# Autodesk Inventor assembly: coil_driver
(part 2 of 3)
- C:\Users\nfitch\Desktop\repos\Imperial\CCMCircuits\CCM_0008_Coil_Driver\cad\RESC1608X446.ipt
- C:\Users\nfitch\Desktop\repos\Imperial\CCMCircuits\CCM_0008_Coil_Driver\cad\RESC1608X447.ipt
- C:\Users\nfitch\Desktop\repos\Imperial\CCMCircuits\CCM_0008_Coil_Driver\cad\RESC1608X448.ipt
- C:\Users\nfitch\Desktop\repos\Imperial\CCMCircuits\CCM_0008_Coil_Driver\cad\RESC1608X449.ipt
- C:\Users\nfitch\Desktop\repos\Imperial\CCMCircuits\CCM_0008_Coil_Driver\cad\RESC1608X450.ipt
- C:\Users\nfitch\Desktop\repos\Imperial\CCMCircuits\CCM_0008_Coil_Driver\cad\RESC1608X451.ipt
- C:\Users\nfitch\Desktop\repos\Imperial\CCMCircuits\CCM_0008_Coil_Driver\cad\RESC1608X452.ipt
- C:\Users\nfitch\Desktop\repos\Imperial\CCMCircuits\CCM_0008_Coil_Driver\cad\RESC1608X453.ipt
- C:\Users\nfitch\Desktop\repos\Imperial\CCMCircuits\CCM_0008_Coil_Driver\cad\RESC1608X454.ipt
- C:\Users\nfitch\Desktop\repos\Imperial\CCMCircuits\CCM_0008_Coil_Driver\cad\RESC1608X455.ipt
- C:\Users\nfitch\Desktop\repos\Imperial\CCMCircuits\CCM_0008_Coil_Driver\cad\RESC1608X456.ipt
- C:\Users\nfitch\Desktop\repos\Imperial\CCMCircuits\CCM_0008_Coil_Driver\cad\RESC1608X457.ipt
- C:\Users\nfitch\Desktop\repos\Imperial\CCMCircuits\CCM_0008_Coil_Driver\cad\RESC1608X458.ipt
- C:\Users\nfitch\Desktop\repos\Imperial\CCMCircuits\CCM_0008_Coil_Driver\cad\RESC1608X459.ipt
- C:\Users\nfitch\Desktop\repos\Imperial\CCMCircuits\CCM_0008_Coil_Driver\cad\RESC1608X460.ipt
- C:\Users\nfitch\Desktop\repos\Imperial\CCMCircuits\CCM_0008_Coil_Driver\cad\RESC1608X461.ipt
- C:\Users\nfitch\Desktop\repos\Imperial\CCMCircuits\CCM_0008_Coil_Driver\cad\RESC1608X462.ipt
- C:\Users\nfitch\Desktop\repos\Imperial\CCMCircuits\CCM_0008_Coil_Driver\cad\RESC1608X463.ipt
- C:\Users\nfitch\Desktop\repos\Imperial\CCMCircuits\CCM_0008_Coil_Driver\cad\RESC1608X464.ipt
- C:\Users\nfitch\Desktop\repos\Imperial\CCMCircuits\CCM_0008_Coil_Driver\cad\RESC1608X465.ipt
- C:\Users\nfitch\Desktop\repos\Imperial\CCMCircuits\CCM_0008_Coil_Driver\cad\RESC1608X466.ipt
- C:\Users\nfitch\Desktop\repos\Imperial\CCMCircuits\CCM_0008_Coil_Driver\cad\RESC1608X467.ipt
- C:\Users\nfitch\Desktop\repos\Imperial\CCMCircuits\CCM_0008_Coil_Driver\cad\RESC1608X468.ipt
- C:\Users\nfitch\Desktop\repos\Imperial\CCMCircuits\CCM_0008_Coil_Driver\cad\RESC1608X469.ipt
- C:\Users\nfitch\Desktop\repos\Imperial\CCMCircuits\CCM_0008_Coil_Driver\cad\RESC1608X470.ipt
- C:\Users\nfitch\Desktop\repos\Imperial\CCMCircuits\CCM_0008_Coil_Driver\cad\RESC1608X471.ipt
- C:\Users\nfitch\Desktop\repos\Imperial\CCMCircuits\CCM_0008_Coil_Driver\cad\RESC1608X472.ipt
- C:\Users\nfitch\Desktop\repos\Imperial\CCMCircuits\CCM_0008_Coil_Driver\cad\RESC1608X473.ipt
- C:\Users\nfitch\Desktop\repos\Imperial\CCMCircuits\CCM_0008_Coil_Driver\cad\RESC1608X474.ipt
- C:\Users\nfitch\Desktop\repos\Imperial\CCMCircuits\CCM_0008_Coil_Driver\cad\RESC1608X475.ipt
- C:\Users\nfitch\Desktop\repos\Imperial\CCMCircuits\CCM_0008_Coil_Driver\cad\RESC1608X476.ipt
- C:\Users\nfitch\Desktop\repos\Imperial\CCMCircuits\CCM_0008_Coil_Driver\cad\RESC1608X477.ipt
- C:\Users\nfitch\Desktop\repos\Imperial\CCMCircuits\CCM_0008_Coil_Driver\cad\RESC1608X478.ipt
- C:\Users\nfitch\Desktop\repos\Imperial\CCMCircuits\CCM_0008_Coil_Driver\cad\RESC1608X479.ipt
- C:\Users\nfitch\Desktop\repos\Imperial\CCMCircuits\CCM_0008_Coil_Driver\cad\RESC1608X480.ipt
- C:\Users\nfitch\Desktop\repos\Imperial\CCMCircuits\CCM_0008_Coil_Driver\cad\RESC1608X481.ipt
- C:\Users\nfitch\Desktop\repos\Imperial\CCMCircuits\CCM_0008_Coil_Driver\cad\RESC1608X482.ipt
- C:\Users\nfitch\Desktop\repos\Imperial\CCMCircuits\CCM_0008_Coil_Driver\cad\RESC1608X483.ipt
- C:\Users\nfitch\Desktop\repos\Imperial\CCMCircuits\CCM_0008_Coil_Driver\cad\RESC1608X484.ipt
- C:\Users\nfitch\Desktop\repos\Imperial\CCMCircuits\CCM_0008_Coil_Driver\cad\RESC1608X485.ipt
- C:\Users\nfitch\Desktop\repos\Imperial\CCMCircuits\CCM_0008_Coil_Driver\cad\RESC1608X486.ipt
- C:\Users\nfitch\Desktop\repos\Imperial\CCMCircuits\CCM_0008_Coil_Driver\cad\RESC1608X487.ipt
- C:\Users\nfitch\Desktop\repos\Imperial\CCMCircuits\CCM_0008_Coil_Driver\cad\RESC1608X488.ipt
- C:\Users\nfitch\Desktop\repos\Imperial\CCMCircuits\CCM_0008_Coil_Driver\cad\RESC1608X489.ipt
- C:\Users\nfitch\Desktop\repos\Imperial\CCMCircuits\CCM_0008_Coil_Driver\cad\RESC1608X490.ipt
- C:\Users\nfitch\Desktop\repos\Imperial\CCMCircuits\CCM_0008_Coil_Driver\cad\RESC1608X491.ipt
- C:\Users\nfitch\Desktop\repos\Imperial\CCMCircuits\CCM_0008_Coil_Driver\cad\RESC1608X492.ipt
- C:\Users\nfitch\Desktop\repos\Imperial\CCMCircuits\CCM_0008_Coil_Driver\cad\RESC1608X493.ipt
- C:\Users\nfitch\Desktop\repos\Imperial\CCMCircuits\CCM_0008_Coil_Driver\cad\RESC1608X494.ipt
- C:\Users\nfitch\Desktop\repos\Imperial\CCMCircuits\CCM_0008_Coil_Driver\cad\RESC1608X495.ipt
- C:\Users\nfitch\Desktop\repos\Imperial\CCMCircuits\CCM_0008_Coil_Driver\cad\RESC1608X496.ipt
- C:\Users\nfitch\Desktop\repos\Imperial\CCMCircuits\CCM_0008_Coil_Driver\cad\RESC1608X497.ipt
- C:\Users\nfitch\Desktop\repos\Imperial\CCMCircuits\CCM_0008_Coil_Driver\cad\RESC1608X498.ipt
- C:\Users\nfitch\Desktop\repos\Imperial\CCMCircuits\CCM_0008_Coil_Driver\cad\RESC1608X499.ipt
- C:\Users\nfitch\Desktop\repos\Imperial\CCMCircuits\CCM_0008_Coil_Driver\cad\RESC1608X500.ipt
- C:\Users\nfitch\Desktop\repos\Imperial\CCMCircuits\CCM_0008_Coil_Driver\cad\RESC1608X501.ipt
- C:\Users\nfitch\Desktop\repos\Imperial\CCMCircuits\CCM_0008_Coil_Driver\cad\RESC1608X502.ipt
- C:\Users\nfitch\Desktop\repos\Imperial\CCMCircuits\CCM_0008_Coil_Driver\cad\RESC1608X503.ipt
- C:\Users\nfitch\Desktop\repos\Imperial\CCMCircuits\CCM_0008_Coil_Driver\cad\RESC1608X504.ipt
- C:\Users\nfitch\Desktop\repos\Imperial\CCMCircuits\CCM_0008_Coil_Driver\cad\RESC1608X505.ipt
- C:\Users\nfitch\Desktop\repos\Imperial\CCMCircuits\CCM_0008_Coil_Driver\cad\RESC1608X506.ipt
- C:\Users\nfitch\Desktop\repos\Imperial\CCMCircuits\CCM_0008_Coil_Driver\cad\RESC1608X507.ipt
- C:\Users\nfitch\Desktop\repos\Imperial\CCMCircuits\CCM_0008_Coil_Driver\cad\RESC1608X508.ipt
- C:\Users\nfitch\Desktop\repos\Imperial\CCMCircuits\CCM_0008_Coil_Driver\cad\RESC1608X509.ipt
- C:\Users\nfitch\Desktop\repos\Imperial\CCMCircuits\CCM_0008_Coil_Driver\cad\RESC1608X510.ipt
- C:\Users\nfitch\Desktop\repos\Imperial\CCMCircuits\CCM_0008_Coil_Driver\cad\RESC1608X511.ipt
- C:\Users\nfitch\Desktop\repos\Imperial\CCMCircuits\CCM_0008_Coil_Driver\cad\RESC1608X512.ipt
- C:\Users\nfitch\Desktop\repos\Imperial\CCMCircuits\CCM_0008_Coil_Driver\cad\RESC1608X513.ipt
- C:\Users\nfitch\Desktop\repos\Imperial\CCMCircuits\CCM_0008_Coil_Driver\cad\RESC1608X514.ipt
- C:\Users\nfitch\Desktop\repos\Imperial\CCMCircuits\CCM_0008_Coil_Driver\cad\SOD3715X136.ipt
- C:\Users\nfitch\Desktop\repos\Imperial\CCMCircuits\CCM_0008_Coil_Driver\cad\SOD3715X137.ipt
- C:\Users\nfitch\Desktop\repos\Imperial\CCMCircuits\CCM_0008_Coil_Driver\cad\SOD3715X135.ipt
- C:\Users\nfitch\Desktop\repos\Imperial\CCMCircuits\CCM_0008_Coil_Driver\cad\SOT95P237X112-005.ipt
- C:\Users\nfitch\Desktop\repos\Imperial\CCMCircuits\CCM_0008_Coil_Driver\cad\SOT95P237X112-006.ipt
- C:\Users\nfitch\Desktop\repos\Imperial\CCMCircuits\CCM_0008_Coil_Driver\cad\SOT95P237X112-3.ipt
- C:\Users\nfitch\Desktop\repos\Imperial\CCMCircuits\CCM_0008_Coil_Driver\cad\SOT95P237X112-004.ipt
- C:\Users\nfitch\Desktop\repos\Imperial\CCMCircuits\CCM_0008_Coil_Driver\cad\SOD3715X138.ipt
- C:\Users\nfitch\Desktop\repos\Imperial\CCMCircuits\CCM_0008_Coil_Driver\cad\SOD3715X139.ipt
- C:\Users\nfitch\Desktop\repos\Imperial\CCMCircuits\CCM_0008_Coil_Driver\cad\SOD3715X140.ipt
- C:\Users\nfitch\Desktop\repos\Imperial\CCMCircuits\CCM_0008_Coil_Driver\cad\SOD3715X141.ipt
- C:\Users\nfitch\Desktop\repos\Imperial\CCMCircuits\CCM_0008_Coil_Driver\cad\SOD3715X142.ipt
- C:\Users\nfitch\Desktop\repos\Imperial\CCMCircuits\CCM_0008_Coil_Driver\cad\SOD3715X143.ipt
- C:\Users\nfitch\Desktop\repos\Imperial\CCMCircuits\CCM_0008_Coil_Driver\cad\SOD3715X144.ipt
- C:\Users\nfitch\Desktop\repos\Imperial\CCMCircuits\CCM_0008_Coil_Driver\cad\SOD3715X145.ipt
- C:\Users\nfitch\Desktop\repos\Imperial\CCMCircuits\CCM_0008_Coil_Driver\cad\SOD3715X146.ipt
- C:\Users\nfitch\Desktop\repos\Imperial\CCMCircuits\CCM_0008_Coil_Driver\cad\SOD3715X147.ipt
- C:\Users\nfitch\Desktop\repos\Imperial\CCMCircuits\CCM_0008_Coil_Driver\cad\SOD3715X148.ipt
- C:\Users\nfitch\Desktop\repos\Imperial\CCMCircuits\CCM_0008_Coil_Driver\cad\SOD3715X149.ipt
- C:\Users\nfitch\Desktop\repos\Imperial\CCMCircuits\CCM_0008_Coil_Driver\cad\SOD3715X150.ipt
- C:\Users\nfitch\Desktop\repos\Imperial\CCMCircuits\CCM_0008_Coil_Driver\cad\SOD3715X151.ipt
- C:\Users\nfitch\Desktop\repos\Imperial\CCMCircuits\CCM_0008_Coil_Driver\cad\SOD3715X152.ipt
- C:\Users\nfitch\Desktop\repos\Imperial\CCMCircuits\CCM_0008_Coil_Driver\cad\Component_1.ipt
- C:\Users\nfitch\Desktop\repos\Imperial\CCMCircuits\CCM_0008_Coil_Driver\cad\Component_2.ipt
- C:\Users\nfitch\Desktop\repos\Imperial\CCMCircuits\CCM_0008_Coil_Driver\cad\Component_003.ipt
- C:\Users\nfitch\Desktop\repos\Imperial\CCMCircuits\CCM_0008_Coil_Driver\cad\Component_004.ipt
- C:\Users\nfitch\Desktop\repos\Imperial\CCMCircuits\CCM_0008_Coil_Driver\cad\SOIC127P600X175-009.ipt
- C:\Users\nfitch\Desktop\repos\Imperial\CCMCircuits\CCM_0008_Coil_Driver\cad\SOIC127P600X175-016.ipt
- C:\Users\nfitch\Desktop\repos\Imperial\CCMCircuits\CCM_0008_Coil_Driver\cad\SOIC127P600X175-010.ipt
- C:\Users\nfitch\Desktop\repos\Imperial\CCMCircuits\CCM_0008_Coil_Driver\cad\SOIC127P600X175-015.ipt
- C:\Users\nfitch\Desktop\repos\Imperial\CCMCircuits\CCM_0008_Coil_Driver\cad\SOIC127P600X175-011.ipt
- C:\Users\nfitch\Desktop\repos\Imperial\CCMCircuits\CCM_0008_Coil_Driver\cad\SOIC127P600X175-012.ipt
- C:\Users\nfitch\Desktop\repos\Imperial\CCMCircuits\CCM_0008_Coil_Driver\cad\SOIC127P600X175-8.ipt
- C:\Users\nfitch\Desktop\repos\Imperial\CCMCircuits\CCM_0008_Coil_Driver\cad\SOIC127P600X175-013.ipt
- C:\Users\nfitch\Desktop\repos\Imperial\CCMCircuits\CCM_0008_Coil_Driver\cad\SOIC127P600X175-014.ipt
- C:\Users\nfitch\Desktop\repos\Imperial\CCMCircuits\CCM_0008_Coil_Driver\cad\SOIC127P600X175-017.ipt
- C:\Users\nfitch\Desktop\repos\Imperial\CCMCircuits\CCM_0008_Coil_Driver\cad\SOIC127P600X175-018.ipt
- C:\Users\nfitch\Desktop\repos\Imperial\CCMCircuits\CCM_0008_Coil_Driver\cad\SOIC127P600X175-019.ipt
- C:\Users\nfitch\Desktop\repos\Imperial\CCMCircuits\CCM_0008_Coil_Driver\cad\SOIC127P600X175-020.ipt
- C:\Users\nfitch\Desktop\repos\Imperial\CCMCircuits\CCM_0008_Coil_Driver\cad\SOIC127P600X175-021.ipt
- C:\Users\nfitch\Desktop\repos\Imperial\CCMCircuits\CCM_0008_Coil_Driver\cad\SOIC127P600X175-022.ipt
- C:\Users\nfitch\Desktop\repos\Imperial\CCMCircuits\CCM_0008_Coil_Driver\cad\SOIC127P600X175-023.ipt
- C:\Users\nfitch\Desktop\repos\Imperial\CCMCircuits\CCM_0008_Coil_Driver\cad\SOIC127P600X175-024.ipt
- C:\Users\nfitch\Desktop\repos\Imperial\CCMCircuits\CCM_0008_Coil_Driver\cad\SOIC127P600X175-025.ipt
- C:\Users\nfitch\Desktop\repos\Imperial\CCMCircuits\CCM_0008_Coil_Driver\cad\SOIC127P600X175-026.ipt
- C:\Users\nfitch\Desktop\repos\Imperial\CCMCircuits\CCM_0008_Coil_Driver\cad\SOIC127P600X175-027.ipt
- C:\Users\nfitch\Desktop\repos\Imperial\CCMCircuits\CCM_0008_Coil_Driver\cad\SOIC127P600X175-028.ipt
- C:\Users\nfitch\Desktop\repos\Imperial\CCMCircuits\CCM_0008_Coil_Driver\cad\SOIC127P600X175-029.ipt
- C:\Users\nfitch\Desktop\repos\Imperial\CCMCircuits\CCM_0008_Coil_Driver\cad\SOIC127P600X175-030.ipt
- C:\Users\nfitch\Desktop\repos\Imperial\CCMCircuits\CCM_0008_Coil_Driver\cad\SOIC127P600X175-031.ipt
- C:\Users\nfitch\Desktop\repos\Imperial\CCMCircuits\CCM_0008_Coil_Driver\cad\SOIC127P600X175-032.ipt
- C:\Users\nfitch\Desktop\repos\Imperial\CCMCircuits\CCM_0008_Coil_Driver\cad\SOIC127P600X175-033.ipt
- C:\Users\nfitch\Desktop\repos\Imperial\CCMCircuits\CCM_0008_Coil_Driver\cad\SOIC127P600X175-034.ipt
- C:\Users\nfitch\Desktop\repos\Imperial\CCMCircuits\CCM_0008_Coil_Driver\cad\SOIC127P600X175-035.ipt
- C:\Users\nfitch\Desktop\repos\Imperial\CCMCircuits\CCM_0008_Coil_Driver\cad\SOIC127P600X175-036.ipt
- C:\Users\nfitch\Desktop\repos\Imperial\CCMCircuits\CCM_0008_Coil_Driver\cad\SOIC127P600X175-037.ipt
- C:\Users\nfitch\Desktop\repos\Imperial\CCMCircuits\CCM_0008_Coil_Driver\cad\SOIC127P600X175-038.ipt
- C:\Users\nfitch\Desktop\repos\Imperial\CCMCircuits\CCM_0008_Coil_Driver\cad\SOIC127P600X175-039.ipt
- C:\Users\nfitch\Desktop\repos\Imperial\CCMCircuits\CCM_0008_Coil_Driver\cad\SOIC127P600X175-040.ipt
- C:\Users\nfitch\Desktop\repos\Imperial\CCMCircuits\CCM_0008_Coil_Driver\cad\SOIC127P600X175-041.ipt
- C:\Users\nfitch\Desktop\repos\Imperial\CCMCircuits\CCM_0008_Coil_Driver\cad\SOIC127P600X175-042.ipt
- C:\Users\nfitch\Desktop\repos\Imperial\CCMCircuits\CCM_0008_Coil_Driver\cad\SOIC127P600X175-043.ipt
- C:\Users\nfitch\Desktop\repos\Imperial\CCMCircuits\CCM_0008_Coil_Driver\cad\SOIC127P600X175-044.ipt
- C:\Users\nfitch\Desktop\repos\Imperial\CCMCircuits\CCM_0008_Coil_Driver\cad\SOIC127P600X175-045.ipt
- C:\Users\nfitch\Desktop\repos\Imperial\CCMCircuits\CCM_0008_Coil_Driver\cad\SOIC127P600X175-046.ipt
- C:\Users\nfitch\Desktop\repos\Imperial\CCMCircuits\CCM_0008_Coil_Driver\cad\SOIC127P600X175-047.ipt
- C:\Users\nfitch\Desktop\repos\Imperial\CCMCircuits\CCM_0008_Coil_Driver\cad\SOIC127P600X175-048.ipt
- C:\Users\nfitch\Desktop\repos\Imperial\CCMCircuits\CCM_0008_Coil_Driver\cad\SOIC127P600X175-049.ipt
- C:\Users\nfitch\Desktop\repos\Imperial\CCMCircuits\CCM_0008_Coil_Driver\cad\SOIC127P600X175-050.ipt
- C:\Users\nfitch\Desktop\repos\Imperial\CCMCircuits\CCM_0008_Coil_Driver\cad\SOIC127P600X175-051.ipt
- C:\Users\nfitch\Desktop\repos\Imperial\CCMCircuits\CCM_0008_Coil_Driver\cad\SOIC127P600X175-052.ipt
- C:\Users\nfitch\Desktop\repos\Imperial\CCMCircuits\CCM_0008_Coil_Driver\cad\SOIC127P600X175-053.ipt
- C:\Users\nfitch\Desktop\repos\Imperial\CCMCircuits\CCM_0008_Coil_Driver\cad\SOIC127P600X175-054.ipt
- C:\Users\nfitch\Desktop\repos\Imperial\CCMCircuits\CCM_0008_Coil_Driver\cad\SOIC127P600X175-055.ipt
- C:\Users\nfitch\Desktop\repos\Imperial\CCMCircuits\CCM_0008_Coil_Driver\cad\SOIC127P600X175-056.ipt
- C:\Users\nfitch\Desktop\repos\Imperial\CCMCircuits\CCM_0008_Coil_Driver\cad\SOIC127P600X175-057.ipt
- C:\Users\nfitch\Desktop\repos\Imperial\CCMCircuits\CCM_0008_Coil_Driver\cad\SOIC127P600X175-058.ipt
- C:\Users\nfitch\Desktop\repos\Imperial\CCMCircuits\CCM_0008_Coil_Driver\cad\SOIC127P600X175-059.ipt
- C:\Users\nfitch\Desktop\repos\Imperial\CCMCircuits\CCM_0008_Coil_Driver\cad\SOIC127P600X175-060.ipt
- C:\Users\nfitch\Desktop\repos\Imperial\CCMCircuits\CCM_0008_Coil_Driver\cad\SOIC127P600X175-061.ipt
- C:\Users\nfitch\Desktop\repos\Imperial\CCMCircuits\CCM_0008_Coil_Driver\cad\SOIC127P600X175-062.ipt
- C:\Users\nfitch\Desktop\repos\Imperial\CCMCircuits\CCM_0008_Coil_Driver\cad\SOIC127P600X175-063.ipt
- C:\Users\nfitch\Desktop\repos\Imperial\CCMCircuits\CCM_0008_Coil_Driver\cad\SOIC127P600X175-064.ipt
- C:\Users\nfitch\Desktop\repos\Imperial\CCMCircuits\CCM_0008_Coil_Driver\cad\SOIC127P600X175-065.ipt
- C:\Users\nfitch\Desktop\repos\Imperial\CCMCircuits\CCM_0008_Coil_Driver\cad\SOIC127P600X175-066.ipt
- C:\Users\nfitch\Desktop\repos\Imperial\CCMCircuits\CCM_0008_Coil_Driver\cad\SOIC127P600X175-067.ipt
- C:\Users\nfitch\Desktop\repos\Imperial\CCMCircuits\CCM_0008_Coil_Driver\cad\SOIC127P600X175-068.ipt
- C:\Users\nfitch\Desktop\repos\Imperial\CCMCircuits\CCM_0008_Coil_Driver\cad\SOIC127P600X175-069.ipt
- C:\Users\nfitch\Desktop\repos\Imperial\CCMCircuits\CCM_0008_Coil_Driver\cad\SOIC127P600X175-070.ipt
- C:\Users\nfitch\Desktop\repos\Imperial\CCMCircuits\CCM_0008_Coil_Driver\cad\SOIC127P600X175-071.ipt
- C:\Users\nfitch\Desktop\repos\Imperial\CCMCircuits\CCM_0008_Coil_Driver\cad\SOIC127P600X175-072.ipt
- C:\Users\nfitch\Desktop\repos\Imperial\CCMCircuits\CCM_0008_Coil_Driver\cad\SOIC127P600X175-073.ipt
- C:\Users\nfitch\Desktop\repos\Imperial\CCMCircuits\CCM_0008_Coil_Driver\cad\SOIC127P600X175-074.ipt
- C:\Users\nfitch\Desktop\repos\Imperial\CCMCircuits\CCM_0008_Coil_Driver\cad\SOIC127P600X175-075.ipt
- C:\Users\nfitch\Desktop\repos\Imperial\CCMCircuits\CCM_0008_Coil_Driver\cad\SOIC127P600X175-076.ipt
- C:\Users\nfitch\Desktop\repos\Imperial\CCMCircuits\CCM_0008_Coil_Driver\cad\SOIC127P600X175-077.ipt
- C:\Users\nfitch\Desktop\repos\Imperial\CCMCircuits\CCM_0008_Coil_Driver\cad\SOIC127P600X175-078.ipt
- C:\Users\nfitch\Desktop\repos\Imperial\CCMCircuits\CCM_0008_Coil_Driver\cad\SOIC127P600X175-079.ipt
- C:\Users\nfitch\Desktop\repos\Imperial\CCMCircuits\CCM_0008_Coil_Driver\cad\SOIC127P600X175-080.ipt
- C:\Users\nfitch\Desktop\repos\Imperial\CCMCircuits\CCM_0008_Coil_Driver\cad\SOIC127P600X175-081.ipt
- C:\Users\nfitch\Desktop\repos\Imperial\CCMCircuits\CCM_0008_Coil_Driver\cad\SOIC127P600X175-082.ipt
- C:\Users\nfitch\Desktop\repos\Imperial\CCMCircuits\CCM_0008_Coil_Driver\cad\SOIC127P600X175-083.ipt
- C:\Users\nfitch\Desktop\repos\Imperial\CCMCircuits\CCM_0008_Coil_Driver\cad\SOIC127P600X175-084.ipt
- C:\Users\nfitch\Desktop\repos\Imperial\CCMCircuits\CCM_0008_Coil_Driver\cad\SOIC127P600X175-085.ipt
- C:\Users\nfitch\Desktop\repos\Imperial\CCMCircuits\CCM_0008_Coil_Driver\cad\SOIC127P600X175-086.ipt
- C:\Users\nfitch\Desktop\repos\Imperial\CCMCircuits\CCM_0008_Coil_Driver\cad\SOIC127P600X175-087.ipt
- C:\Users\nfitch\Desktop\repos\Imperial\CCMCircuits\CCM_0008_Coil_Driver\cad\SOIC127P600X175-088.ipt
- C:\Users\nfitch\Desktop\repos\Imperial\CCMCircuits\CCM_0008_Coil_Driver\cad\SOIC127P600X175-089.ipt
- C:\Users\nfitch\Desktop\repos\Imperial\CCMCircuits\CCM_0008_Coil_Driver\cad\SOIC127P600X175-090.ipt
- C:\Users\nfitch\Desktop\repos\Imperial\CCMCircuits\CCM_0008_Coil_Driver\cad\SOIC127P600X175-091.ipt
- C:\Users\nfitch\Desktop\repos\Imperial\CCMCircuits\CCM_0008_Coil_Driver\cad\SOIC127P600X175-092.ipt
- C:\Users\nfitch\Desktop\repos\Imperial\CCMCircuits\CCM_0008_Coil_Driver\cad\SOIC127P600X175-093.ipt
- C:\Users\nfitch\Desktop\repos\Imperial\CCMCircuits\CCM_0008_Coil_Driver\cad\SOIC127P600X175-094.ipt
- C:\Users\nfitch\Desktop\repos\Imperial\CCMCircuits\CCM_0008_Coil_Driver\cad\SOIC127P600X175-095.ipt
- C:\Users\nfitch\Desktop\repos\Imperial\CCMCircuits\CCM_0008_Coil_Driver\cad\SOIC127P600X175-096.ipt
- C:\Users\nfitch\Desktop\repos\Imperial\CCMCircuits\CCM_0008_Coil_Driver\cad\SOIC127P600X175-097.ipt
- C:\Users\nfitch\Desktop\repos\Imperial\CCMCircuits\CCM_0008_Coil_Driver\cad\SOIC127P600X175-098.ipt
- C:\Users\nfitch\Desktop\repos\Imperial\CCMCircuits\CCM_0008_Coil_Driver\cad\SOIC127P600X175-099.ipt
- C:\Users\nfitch\Desktop\repos\Imperial\CCMCircuits\CCM_0008_Coil_Driver\cad\SOIC127P600X175-100.ipt
- C:\Users\nfitch\Desktop\repos\Imperial\CCMCircuits\CCM_0008_Coil_Driver\cad\SOIC127P600X175-101.ipt
- C:\Users\nfitch\Desktop\repos\Imperial\CCMCircuits\CCM_0008_Coil_Driver\cad\SOIC127P600X175-102.ipt
- C:\Users\nfitch\Desktop\repos\Imperial\CCMCircuits\CCM_0008_Coil_Driver\cad\SOIC127P600X175-103.ipt
- C:\Users\nfitch\Desktop\repos\Imperial\CCMCircuits\CCM_0008_Coil_Driver\cad\SOIC127P600X175-104.ipt
- C:\Users\nfitch\Desktop\repos\Imperial\CCMCircuits\CCM_0008_Coil_Driver\cad\SOIC127P600X175-105.ipt
- C:\Users\nfitch\Desktop\repos\Imperial\CCMCircuits\CCM_0008_Coil_Driver\cad\SOIC127P600X175-106.ipt
- C:\Users\nfitch\Desktop\repos\Imperial\CCMCircuits\CCM_0008_Coil_Driver\cad\SOIC127P600X175-107.ipt
- C:\Users\nfitch\Desktop\repos\Imperial\CCMCircuits\CCM_0008_Coil_Driver\cad\SOIC127P600X175-108.ipt
- C:\Users\nfitch\Desktop\repos\Imperial\CCMCircuits\CCM_0008_Coil_Driver\cad\SOIC127P600X175-109.ipt
- C:\Users\nfitch\Desktop\repos\Imperial\CCMCircuits\CCM_0008_Coil_Driver\cad\SOIC127P600X175-110.ipt
- C:\Users\nfitch\Desktop\repos\Imperial\CCMCircuits\CCM_0008_Coil_Driver\cad\SOIC127P600X175-111.ipt
- C:\Users\nfitch\Desktop\repos\Imperial\CCMCircuits\CCM_0008_Coil_Driver\cad\SOIC127P600X175-112.ipt
- C:\Users\nfitch\Desktop\repos\Imperial\CCMCircuits\CCM_0008_Coil_Driver\cad\SOIC127P600X175-113.ipt
- C:\Users\nfitch\Desktop\repos\Imperial\CCMCircuits\CCM_0008_Coil_Driver\cad\SOIC127P600X175-114.ipt
- C:\Users\nfitch\Desktop\repos\Imperial\CCMCircuits\CCM_0008_Coil_Driver\cad\SOIC127P600X175-115.ipt
- C:\Users\nfitch\Desktop\repos\Imperial\CCMCircuits\CCM_0008_Coil_Driver\cad\SOIC127P600X175-116.ipt
- C:\Users\nfitch\Desktop\repos\Imperial\CCMCircuits\CCM_0008_Coil_Driver\cad\SOIC127P600X175-117.ipt
- C:\Users\nfitch\Desktop\repos\Imperial\CCMCircuits\CCM_0008_Coil_Driver\cad\SOIC127P600X175-118.ipt
- C:\Users\nfitch\Desktop\repos\Imperial\CCMCircuits\CCM_0008_Coil_Driver\cad\SOIC127P600X175-119.ipt
- C:\Users\nfitch\Desktop\repos\Imperial\CCMCircuits\CCM_0008_Coil_Driver\cad\SOIC127P600X175-120.ipt
- C:\Users\nfitch\Desktop\repos\Imperial\CCMCircuits\CCM_0008_Coil_Driver\cad\SOIC127P600X175-121.ipt
- C:\Users\nfitch\Desktop\repos\Imperial\CCMCircuits\CCM_0008_Coil_Driver\cad\SOIC127P600X175-122.ipt
- C:\Users\nfitch\Desktop\repos\Imperial\CCMCircuits\CCM_0008_Coil_Driver\cad\SOIC127P600X175-123.ipt
- C:\Users\nfitch\Desktop\repos\Imperial\CCMCircuits\CCM_0008_Coil_Driver\cad\SOIC127P600X175-124.ipt
- C:\Users\nfitch\Desktop\repos\Imperial\CCMCircuits\CCM_0008_Coil_Driver\cad\SOIC127P600X175-125.ipt
- C:\Users\nfitch\Desktop\repos\Imperial\CCMCircuits\CCM_0008_Coil_Driver\cad\SOIC127P600X175-126.ipt
- C:\Users\nfitch\Desktop\repos\Imperial\CCMCircuits\CCM_0008_Coil_Driver\cad\SOIC127P600X175-127.ipt
- C:\Users\nfitch\Desktop\repos\Imperial\CCMCircuits\CCM_0008_Coil_Driver\cad\SOIC127P600X175-128.ipt
- C:\Users\nfitch\Desktop\repos\Imperial\CCMCircuits\CCM_0008_Coil_Driver\cad\SOIC127P600X175-129.ipt
- C:\Users\nfitch\Desktop\repos\Imperial\CCMCircuits\CCM_0008_Coil_Driver\cad\SOIC127P600X175-130.ipt
- C:\Users\nfitch\Desktop\repos\Imperial\CCMCircuits\CCM_0008_Coil_Driver\cad\SOIC127P600X175-131.ipt
- C:\Users\nfitch\Desktop\repos\Imperial\CCMCircuits\CCM_0008_Coil_Driver\cad\SOIC127P600X175-132.ipt
- C:\Users\nfitch\Desktop\repos\Imperial\CCMCircuits\CCM_0008_Coil_Driver\cad\SOIC127P600X175-133.ipt
- C:\Users\nfitch\Desktop\repos\Imperial\CCMCircuits\CCM_0008_Coil_Driver\cad\SOIC127P600X175-134.ipt
- C:\Users\nfitch\Desktop\repos\Imperial\CCMCircuits\CCM_0008_Coil_Driver\cad\SOIC127P600X175-135.ipt
- C:\Users\nfitch\Desktop\repos\Imperial\CCMCircuits\CCM_0008_Coil_Driver\cad\SOIC127P600X175-136.ipt
- C:\Users\nfitch\Desktop\repos\Imperial\CCMCircuits\CCM_0008_Coil_Driver\cad\SOIC127P600X175-137.ipt
- C:\Users\nfitch\Desktop\repos\Imperial\CCMCircuits\CCM_0008_Coil_Driver\cad\SOIC127P600X175-138.ipt
- C:\Users\nfitch\Desktop\repos\Imperial\CCMCircuits\CCM_0008_Coil_Driver\cad\SOIC127P600X175-139.ipt
- C:\Users\nfitch\Desktop\repos\Imperial\CCMCircuits\CCM_0008_Coil_Driver\cad\SOIC127P600X175-140.ipt
- C:\Users\nfitch\Desktop\repos\Imperial\CCMCircuits\CCM_0008_Coil_Driver\cad\SOIC127P600X175-141.ipt
- C:\Users\nfitch\Desktop\repos\Imperial\CCMCircuits\CCM_0008_Coil_Driver\cad\SOIC127P600X175-142.ipt
- C:\Users\nfitch\Desktop\repos\Imperial\CCMCircuits\CCM_0008_Coil_Driver\cad\SOIC127P600X175-143.ipt
- C:\Users\nfitch\Desktop\repos\Imperial\CCMCircuits\CCM_0008_Coil_Driver\cad\SOIC127P600X175-144.ipt
- C:\Users\nfitch\Desktop\repos\Imperial\CCMCircuits\CCM_0008_Coil_Driver\cad\SOIC127P600X175-145.ipt
- C:\Users\nfitch\Desktop\repos\Imperial\CCMCircuits\CCM_0008_Coil_Driver\cad\SOIC127P600X175-146.ipt
- C:\Users\nfitch\Desktop\repos\Imperial\CCMCircuits\CCM_0008_Coil_Driver\cad\SOIC127P600X175-147.ipt
- C:\Users\nfitch\Desktop\repos\Imperial\CCMCircuits\CCM_0008_Coil_Driver\cad\SOIC127P600X175-148.ipt
- C:\Users\nfitch\Desktop\repos\Imperial\CCMCircuits\CCM_0008_Coil_Driver\cad\SOIC127P600X175-149.ipt
- C:\Users\nfitch\Desktop\repos\Imperial\CCMCircuits\CCM_0008_Coil_Driver\cad\SOIC127P600X175-150.ipt
- C:\Users\nfitch\Desktop\repos\Imperial\CCMCircuits\CCM_0008_Coil_Driver\cad\SOIC127P600X175-151.ipt
- C:\Users\nfitch\Desktop\repos\Imperial\CCMCircuits\CCM_0008_Coil_Driver\cad\SOIC127P600X175-152.ipt
- C:\Users\nfitch\Desktop\repos\Imperial\CCMCircuits\CCM_0008_Coil_Driver\cad\SOIC127P600X175-153.ipt
- C:\Users\nfitch\Desktop\repos\Imperial\CCMCircuits\CCM_0008_Coil_Driver\cad\SOIC127P600X175-154.ipt
- C:\Users\nfitch\Desktop\repos\Imperial\CCMCircuits\CCM_0008_Coil_Driver\cad\SOIC127P600X175-155.ipt
- C:\Users\nfitch\Desktop\repos\Imperial\CCMCircuits\CCM_0008_Coil_Driver\cad\SOIC127P600X175-156.ipt
- C:\Users\nfitch\Desktop\repos\Imperial\CCMCircuits\CCM_0008_Coil_Driver\cad\SOIC127P600X175-157.ipt
- C:\Users\nfitch\Desktop\repos\Imperial\CCMCircuits\CCM_0008_Coil_Driver\cad\SOIC127P600X175-158.ipt
- C:\Users\nfitch\Desktop\repos\Imperial\CCMCircuits\CCM_0008_Coil_Driver\cad\SOIC127P600X175-159.ipt
- C:\Users\nfitch\Desktop\repos\Imperial\CCMCircuits\CCM_0008_Coil_Driver\cad\SOIC127P600X175-160.ipt
- C:\Users\nfitch\Desktop\repos\Imperial\CCMCircuits\CCM_0008_Coil_Driver\cad\002.ipt
- C:\Users\nfitch\Desktop\repos\Imperial\CCMCircuits\CCM_0008_Coil_Driver\cad\1.ipt
- C:\Users\nfitch\Desktop\repos\Imperial\CCMCircuits\CCM_0008_Coil_Driver\cad\002001.ipt
- C:\Users\nfitch\Desktop\repos\Imperial\CCMCircuits\CCM_0008_Coil_Driver\cad\1001.ipt
- C:\Users\nfitch\Desktop\repos\Imperial\CCMCircuits\CCM_0008_Coil_Driver\cad\002002.ipt
- C:\Users\nfitch\Desktop\repos\Imperial\CCMCircuits\CCM_0008_Coil_Driver\cad\1002.ipt
- C:\Users\nfitch\Desktop\repos\Imperial\CCMCircuits\CCM_0008_Coil_Driver\cad\002003.ipt
- C:\Users\nfitch\Desktop\repos\Imperial\CCMCircuits\CCM_0008_Coil_Driver\cad\1003.ipt
- C:\Users\nfitch\Desktop\repos\Imperial\CCMCircuits\CCM_0008_Coil_Driver\cad\3009P_ASM_Next_assembly_relationship;33256-61701.ipt
- C:\Users\nfitch\Desktop\repos\Imperial\CCMCircuits\CCM_0008_Coil_Driver\cad\RESC1608X515.ipt
- C:\Users\nfitch\Desktop\repos\Imperial\CCMCircuits\CCM_0008_Coil_Driver\cad\RESC1608X516.ipt
- C:\Users\nfitch\Desktop\repos\Imperial\CCMCircuits\CCM_0008_Coil_Driver\cad\RESC1608X517.ipt
- C:\Users\nfitch\Desktop\repos\Imperial\CCMCircuits\CCM_0008_Coil_Driver\cad\RESC1608X518.ipt
- C:\Users\nfitch\Desktop\repos\Imperial\CCMCircuits\CCM_0008_Coil_Driver\cad\RESC1608X519.ipt
- C:\Users\nfitch\Desktop\repos\Imperial\CCMCircuits\CCM_0008_Coil_Driver\cad\RESC1608X520.ipt
- C:\Users\nfitch\Desktop\repos\Imperial\CCMCircuits\CCM_0008_Coil_Driver\cad\RESC1608X521.ipt
- C:\Users\nfitch\Desktop\repos\Imperial\CCMCircuits\CCM_0008_Coil_Driver\cad\RESC1608X522.ipt
- C:\Users\nfitch\Desktop\repos\Imperial\CCMCircuits\CCM_0008_Coil_Driver\cad\RESC1608X523.ipt
- C:\Users\nfitch\Desktop\repos\Imperial\CCMCircuits\CCM_0008_Coil_Driver\cad\RESC1608X524.ipt
- C:\Users\nfitch\Desktop\repos\Imperial\CCMCircuits\CCM_0008_Coil_Driver\cad\RESC1608X525.ipt
- C:\Users\nfitch\Desktop\repos\Imperial\CCMCircuits\CCM_0008_Coil_Driver\cad\RESC1608X526.ipt
- C:\Users\nfitch\Desktop\repos\Imperial\CCMCircuits\CCM_0008_Coil_Driver\cad\RESC1608X527.ipt
- C:\Users\nfitch\Desktop\repos\Imperial\CCMCircuits\CCM_0008_Coil_Driver\cad\RESC1608X528.ipt
- C:\Users\nfitch\Desktop\repos\Imperial\CCMCircuits\CCM_0008_Coil_Driver\cad\RESC1608X529.ipt
- C:\Users\nfitch\Desktop\repos\Imperial\CCMCircuits\CCM_0008_Coil_Driver\cad\RESC1608X530.ipt
- C:\Users\nfitch\Desktop\repos\Imperial\CCMCircuits\CCM_0008_Coil_Driver\cad\RESC1608X531.ipt
- C:\Users\nfitch\Desktop\repos\Imperial\CCMCircuits\CCM_0008_Coil_Driver\cad\RESC1608X532.ipt
- C:\Users\nfitch\Desktop\repos\Imperial\CCMCircuits\CCM_0008_Coil_Driver\cad\RESC1608X533.ipt
- C:\Users\nfitch\Desktop\repos\Imperial\CCMCircuits\CCM_0008_Coil_Driver\cad\RESC1608X534.ipt
- C:\Users\nfitch\Desktop\repos\Imperial\CCMCircuits\CCM_0008_Coil_Driver\cad\RESC1608X535.ipt
- C:\Users\nfitch\Desktop\repos\Imperial\CCMCircuits\CCM_0008_Coil_Driver\cad\RESC1608X536.ipt
- C:\Users\nfitch\Desktop\repos\Imperial\CCMCircuits\CCM_0008_Coil_Driver\cad\RESC1608X537.ipt
- C:\Users\nfitch\Desktop\repos\Imperial\CCMCircuits\CCM_0008_Coil_Driver\cad\RESC1608X538.ipt
- C:\Users\nfitch\Desktop\repos\Imperial\CCMCircuits\CCM_0008_Coil_Driver\cad\RESC1608X539.ipt
- C:\Users\nfitch\Desktop\repos\Imperial\CCMCircuits\CCM_0008_Coil_Driver\cad\RESC1608X540.ipt
- C:\Users\nfitch\Desktop\repos\Imperial\CCMCircuits\CCM_0008_Coil_Driver\cad\RESC1608X541.ipt
- C:\Users\nfitch\Desktop\repos\Imperial\CCMCircuits\CCM_0008_Coil_Driver\cad\RESC1608X542.ipt
- C:\Users\nfitch\Desktop\repos\Imperial\CCMCircuits\CCM_0008_Coil_Driver\cad\RESC1608X543.ipt
- C:\Users\nfitch\Desktop\repos\Imperial\CCMCircuits\CCM_0008_Coil_Driver\cad\RESC1608X544.ipt
- C:\Users\nfitch\Desktop\repos\Imperial\CCMCircuits\CCM_0008_Coil_Driver\cad\RESC1608X545.ipt
- C:\Users\nfitch\Desktop\repos\Imperial\CCMCircuits\CCM_0008_Coil_Driver\cad\RESC1608X546.ipt
- C:\Users\nfitch\Desktop\repos\Imperial\CCMCircuits\CCM_0008_Coil_Driver\cad\RESC1608X547.ipt
- C:\Users\nfitch\Desktop\repos\Imperial\CCMCircuits\CCM_0008_Coil_Driver\cad\RESC1608X548.ipt
- C:\Users\nfitch\Desktop\repos\Imperial\CCMCircuits\CCM_0008_Coil_Driver\cad\RESC1608X549.ipt
- C:\Users\nfitch\Desktop\repos\Imperial\CCMCircuits\CCM_0008_Coil_Driver\cad\3009P_ASM_Next_assembly_relationship;33256-61702.ipt
- C:\Users\nfitch\Desktop\repos\Imperial\CCMCircuits\CCM_0008_Coil_Driver\cad\RESC1608X550.ipt
- C:\Users\nfitch\Desktop\repos\Imperial\CCMCircuits\CCM_0008_Coil_Driver\cad\RESC1608X551.ipt
- C:\Users\nfitch\Desktop\repos\Imperial\CCMCircuits\CCM_0008_Coil_Driver\cad\RESC1608X552.ipt
- C:\Users\nfitch\Desktop\repos\Imperial\CCMCircuits\CCM_0008_Coil_Driver\cad\RESC1608X553.ipt
- C:\Users\nfitch\Desktop\repos\Imperial\CCMCircuits\CCM_0008_Coil_Driver\cad\RESC1608X554.ipt
- C:\Users\nfitch\Desktop\repos\Imperial\CCMCircuits\CCM_0008_Coil_Driver\cad\RESC1608X555.ipt
- C:\Users\nfitch\Desktop\repos\Imperial\CCMCircuits\CCM_0008_Coil_Driver\cad\RESC1608X556.ipt
- C:\Users\nfitch\Desktop\repos\Imperial\CCMCircuits\CCM_0008_Coil_Driver\cad\RESC1608X557.ipt
- C:\Users\nfitch\Desktop\repos\Imperial\CCMCircuits\CCM_0008_Coil_Driver\cad\RESC1608X558.ipt
- C:\Users\nfitch\Desktop\repos\Imperial\CCMCircuits\CCM_0008_Coil_Driver\cad\RESC1608X559.ipt
- C:\Users\nfitch\Desktop\repos\Imperial\CCMCircuits\CCM_0008_Coil_Driver\cad\RESC1608X560.ipt
- C:\Users\nfitch\Desktop\repos\Imperial\CCMCircuits\CCM_0008_Coil_Driver\cad\RESC1608X561.ipt
- C:\Users\nfitch\Desktop\repos\Imperial\CCMCircuits\CCM_0008_Coil_Driver\cad\RESC1608X562.ipt
- C:\Users\nfitch\Desktop\repos\Imperial\CCMCircuits\CCM_0008_Coil_Driver\cad\RESC1608X563.ipt
- C:\Users\nfitch\Desktop\repos\Imperial\CCMCircuits\CCM_0008_Coil_Driver\cad\RESC1608X564.ipt
- C:\Users\nfitch\Desktop\repos\Imperial\CCMCircuits\CCM_0008_Coil_Driver\cad\RESC1608X565.ipt
- C:\Users\nfitch\Desktop\repos\Imperial\CCMCircuits\CCM_0008_Coil_Driver\cad\RESC1608X566.ipt
- C:\Users\nfitch\Desktop\repos\Imperial\CCMCircuits\CCM_0008_Coil_Driver\cad\RESC1608X567.ipt
- C:\Users\nfitch\Desktop\repos\Imperial\CCMCircuits\CCM_0008_Coil_Driver\cad\RESC1608X568.ipt
- C:\Users\nfitch\Desktop\repos\Imperial\CCMCircuits\CCM_0008_Coil_Driver\cad\RESC1608X569.ipt
- C:\Users\nfitch\Desktop\repos\Imperial\CCMCircuits\CCM_0008_Coil_Driver\cad\RESC1608X570.ipt
- C:\Users\nfitch\Desktop\repos\Imperial\CCMCircuits\CCM_0008_Coil_Driver\cad\RESC1608X571.ipt
- C:\Users\nfitch\Desktop\repos\Imperial\CCMCircuits\CCM_0008_Coil_Driver\cad\RESC1608X572.ipt
- C:\Users\nfitch\Desktop\repos\Imperial\CCMCircuits\CCM_0008_Coil_Driver\cad\RESC1608X573.ipt
- C:\Users\nfitch\Desktop\repos\Imperial\CCMCircuits\CCM_0008_Coil_Driver\cad\RESC1608X574.ipt
- C:\Users\nfitch\Desktop\repos\Imperial\CCMCircuits\CCM_0008_Coil_Driver\cad\RESC1608X575.ipt
- C:\Users\nfitch\Desktop\repos\Imperial\CCMCircuits\CCM_0008_Coil_Driver\cad\RESC1608X576.ipt
- C:\Users\nfitch\Desktop\repos\Imperial\CCMCircuits\CCM_0008_Coil_Driver\cad\RESC1608X577.ipt
- C:\Users\nfitch\Desktop\repos\Imperial\CCMCircuits\CCM_0008_Coil_Driver\cad\RESC1608X578.ipt
- C:\Users\nfitch\Desktop\repos\Imperial\CCMCircuits\CCM_0008_Coil_Driver\cad\RESC1608X579.ipt
- C:\Users\nfitch\Desktop\repos\Imperial\CCMCircuits\CCM_0008_Coil_Driver\cad\RESC1608X580.ipt
- C:\Users\nfitch\Desktop\repos\Imperial\CCMCircuits\CCM_0008_Coil_Driver\cad\RESC1608X581.ipt
- C:\Users\nfitch\Desktop\repos\Imperial\CCMCircuits\CCM_0008_Coil_Driver\cad\RESC1608X582.ipt
- C:\Users\nfitch\Desktop\repos\Imperial\CCMCircuits\CCM_0008_Coil_Driver\cad\RESC1608X583.ipt
- C:\Users\nfitch\Desktop\repos\Imperial\CCMCircuits\CCM_0008_Coil_Driver\cad\RESC1608X584.ipt
- C:\Users\nfitch\Desktop\repos\Imperial\CCMCircuits\CCM_0008_Coil_Driver\cad\RESC1608X585.ipt
- C:\Users\nfitch\Desktop\repos\Imperial\CCMCircuits\CCM_0008_Coil_Driver\cad\RESC1608X586.ipt
- C:\Users\nfitch\Desktop\repos\Imperial\CCMCircuits\CCM_0008_Coil_Driver\cad\RESC1608X587.ipt
- C:\Users\nfitch\Desktop\repos\Imperial\CCMCircuits\CCM_0008_Coil_Driver\cad\RESC1608X588.ipt
- C:\Users\nfitch\Desktop\repos\Imperial\CCMCircuits\CCM_0008_Coil_Driver\cad\RESC1608X589.ipt
- C:\Users\nfitch\Desktop\repos\Imperial\CCMCircuits\CCM_0008_Coil_Driver\cad\RESC1608X590.ipt
- C:\Users\nfitch\Desktop\repos\Imperial\CCMCircuits\CCM_0008_Coil_Driver\cad\RESC1608X591.ipt
- C:\Users\nfitch\Desktop\repos\Imperial\CCMCircuits\CCM_0008_Coil_Driver\cad\RESC1608X592.ipt
- C:\Users\nfitch\Desktop\repos\Imperial\CCMCircuits\CCM_0008_Coil_Driver\cad\RESC1608X593.ipt
- C:\Users\nfitch\Desktop\repos\Imperial\CCMCircuits\CCM_0008_Coil_Driver\cad\RESC1608X594.ipt
- C:\Users\nfitch\Desktop\repos\Imperial\CCMCircuits\CCM_0008_Coil_Driver\cad\RESC1608X595.ipt
- C:\Users\nfitch\Desktop\repos\Imperial\CCMCircuits\CCM_0008_Coil_Driver\cad\RESC1608X596.ipt
- C:\Users\nfitch\Desktop\repos\Imperial\CCMCircuits\CCM_0008_Coil_Driver\cad\RESC1608X597.ipt
- C:\Users\nfitch\Desktop\repos\Imperial\CCMCircuits\CCM_0008_Coil_Driver\cad\RESC1608X598.ipt
- C:\Users\nfitch\Desktop\repos\Imperial\CCMCircuits\CCM_0008_Coil_Driver\cad\RESC1608X599.ipt
- C:\Users\nfitch\Desktop\repos\Imperial\CCMCircuits\CCM_0008_Coil_Driver\cad\RESC1608X600.ipt
- C:\Users\nfitch\Desktop\repos\Imperial\CCMCircuits\CCM_0008_Coil_Driver\cad\RESC1608X601.ipt
- C:\Users\nfitch\Desktop\repos\Imperial\CCMCircuits\CCM_0008_Coil_Driver\cad\RESC1608X602.ipt
- C:\Users\nfitch\Desktop\repos\Imperial\CCMCircuits\CCM_0008_Coil_Driver\cad\RESC1608X603.ipt
- C:\Users\nfitch\Desktop\repos\Imperial\CCMCircuits\CCM_0008_Coil_Driver\cad\RESC1608X604.ipt
- C:\Users\nfitch\Desktop\repos\Imperial\CCMCircuits\CCM_0008_Coil_Driver\cad\RESC1608X605.ipt
- C:\Users\nfitch\Desktop\repos\Imperial\CCMCircuits\CCM_0008_Coil_Driver\cad\RESC1608X606.ipt
- C:\Users\nfitch\Desktop\repos\Imperial\CCMCircuits\CCM_0008_Coil_Driver\cad\RESC1608X607.ipt
- C:\Users\nfitch\Desktop\repos\Imperial\CCMCircuits\CCM_0008_Coil_Driver\cad\RESC1608X608.ipt
- C:\Users\nfitch\Desktop\repos\Imperial\CCMCircuits\CCM_0008_Coil_Driver\cad\RESC1608X609.ipt
- C:\Users\nfitch\Desktop\repos\Imperial\CCMCircuits\CCM_0008_Coil_Driver\cad\RESC1608X610.ipt
- C:\Users\nfitch\Desktop\repos\Imperial\CCMCircuits\CCM_0008_Coil_Driver\cad\RESC1608X611.ipt
- C:\Users\nfitch\Desktop\repos\Imperial\CCMCircuits\CCM_0008_Coil_Driver\cad\RESC1608X612.ipt
- C:\Users\nfitch\Desktop\repos\Imperial\CCMCircuits\CCM_0008_Coil_Driver\cad\RESC1608X613.ipt
- C:\Users\nfitch\Desktop\repos\Imperial\CCMCircuits\CCM_0008_Coil_Driver\cad\RESC1608X614.ipt
- C:\Users\nfitch\Desktop\repos\Imperial\CCMCircuits\CCM_0008_Coil_Driver\cad\RESC1608X615.ipt
- C:\Users\nfitch\Desktop\repos\Imperial\CCMCircuits\CCM_0008_Coil_Driver\cad\RESC1608X616.ipt
- C:\Users\nfitch\Desktop\repos\Imperial\CCMCircuits\CCM_0008_Coil_Driver\cad\RESC1608X617.ipt
- C:\Users\nfitch\Desktop\repos\Imperial\CCMCircuits\CCM_0008_Coil_Driver\cad\RESC1608X618.ipt
- C:\Users\nfitch\Desktop\repos\Imperial\CCMCircuits\CCM_0008_Coil_Driver\cad\RESC1608X619.ipt
- C:\Users\nfitch\Desktop\repos\Imperial\CCMCircuits\CCM_0008_Coil_Driver\cad\RESC1608X620.ipt
- C:\Users\nfitch\Desktop\repos\Imperial\CCMCircuits\CCM_0008_Coil_Driver\cad\RESC1608X621.ipt
- C:\Users\nfitch\Desktop\repos\Imperial\CCMCircuits\CCM_0008_Coil_Driver\cad\RESC1608X622.ipt
- C:\Users\nfitch\Desktop\repos\Imperial\CCMCircuits\CCM_0008_Coil_Driver\cad\RESC1608X623.ipt
- C:\Users\nfitch\Desktop\repos\Imperial\CCMCircuits\CCM_0008_Coil_Driver\cad\RESC1608X624.ipt
- C:\Users\nfitch\Desktop\repos\Imperial\CCMCircuits\CCM_0008_Coil_Driver\cad\RESC1608X625.ipt
- C:\Users\nfitch\Desktop\repos\Imperial\CCMCircuits\CCM_0008_Coil_Driver\cad\RESC1608X626.ipt
- C:\Users\nfitch\Desktop\repos\Imperial\CCMCircuits\CCM_0008_Coil_Driver\cad\RESC1608X627.ipt
- C:\Users\nfitch\Desktop\repos\Imperial\CCMCircuits\CCM_0008_Coil_Driver\cad\RESC1608X628.ipt
- C:\Users\nfitch\Desktop\repos\Imperial\CCMCircuits\CCM_0008_Coil_Driver\cad\RESC1608X629.ipt
- C:\Users\nfitch\Desktop\repos\Imperial\CCMCircuits\CCM_0008_Coil_Driver\cad\RESC1608X630.ipt
- C:\Users\nfitch\Desktop\repos\Imperial\CCMCircuits\CCM_0008_Coil_Driver\cad\RESC1608X631.ipt
- C:\Users\nfitch\Desktop\repos\Imperial\CCMCircuits\CCM_0008_Coil_Driver\cad\RESC1608X632.ipt
- C:\Users\nfitch\Desktop\repos\Imperial\CCMCircuits\CCM_0008_Coil_Driver\cad\RESC1608X633.ipt
- C:\Users\nfitch\Desktop\repos\Imperial\CCMCircuits\CCM_0008_Coil_Driver\cad\RESC1608X634.ipt
- C:\Users\nfitch\Desktop\repos\Imperial\CCMCircuits\CCM_0008_Coil_Driver\cad\RESC1608X635.ipt
- C:\Users\nfitch\Desktop\repos\Imperial\CCMCircuits\CCM_0008_Coil_Driver\cad\RESC1608X636.ipt
- C:\Users\nfitch\Desktop\repos\Imperial\CCMCircuits\CCM_0008_Coil_Driver\cad\RESC1608X637.ipt
- C:\Users\nfitch\Desktop\repos\Imperial\CCMCircuits\CCM_0008_Coil_Driver\cad\RESC1608X638.ipt
- C:\Users\nfitch\Desktop\repos\Imperial\CCMCircuits\CCM_0008_Coil_Driver\cad\RESC1608X639.ipt
- C:\Users\nfitch\Desktop\repos\Imperial\CCMCircuits\CCM_0008_Coil_Driver\cad\RESC1608X640.ipt
- C:\Users\nfitch\Desktop\repos\Imperial\CCMCircuits\CCM_0008_Coil_Driver\cad\RESC1608X641.ipt
- C:\Users\nfitch\Desktop\repos\Imperial\CCMCircuits\CCM_0008_Coil_Driver\cad\RESC1608X642.ipt